# Autodesk Inventor assembly: Harbor Freight 10 in Wheel
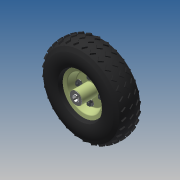
[picture p0: Inventor's stored thumbnail of the model, 180x180]
Saved by Autodesk Inventor 2018 (Build 220112000, 112)
## iProperties
Created: 2017-12-16
Part Number: Harbor Freight 10 in Wheel
Document SubType Name: Assembly
Designer: David
Author: David
## Documents named in this file (8)
- C:\Users\David\Documents\Inventor\Master\RC Car\Harbor Freight 10 in Wheel\Harbor Freight 10 in Wheel.iam
- C:\Users\David\Documents\Inventor\Master\RC Car\Harbor Freight 10 in Wheel\Hub Outer.ipt
- C:\Users\David\Documents\Inventor\Master\RC Car\Harbor Freight 10 in Wheel\Bolt M8x14mm.ipt
- C:\Users\David\Documents\Inventor\Master\RC Car\Harbor Freight 10 in Wheel\Nut M8.ipt
- C:\Users\David\Documents\Inventor\Master\RC Car\Harbor Freight 10 in Wheel\Washer Flat M8.ipt
- C:\Users\David\Documents\Inventor\Master\RC Car\Harbor Freight 10 in Wheel\Tire.ipt
- C:\Users\David\Documents\Inventor\Master\RC Car\Harbor Freight 10 in Wheel\Bearing.ipt
- C:\Users\David\Documents\Inventor\Master\RC Car\Harbor Freight 10 in Wheel\Hub Inner No Holes.ipt
## Components (21 placed, 7 different names)
1. Hub Inner No Holes:1 — Mate:1, Mate:2, Mate:3, Insert:13, Insert:14, Insert:15, Insert:16, Mate:6, Mate:7, Mate:8
2. Hub Outer:1 — Mate:1, Mate:2, Mate:3, Mate:4, Mate:9
3. Bolt M8x14mm:1 — Insert:1
4. Nut M8:1 — Insert:3
5. Washer Flat M8:1 — Insert:2, Insert:3, Insert:14
6. Washer Flat M8:2 — Insert:1, Insert:2
7. Bolt M8x14mm:2
8. Nut M8:2
9. Washer Flat M8:3 — Insert:13
10. Washer Flat M8:4
11. Bolt M8x14mm:3
12. Nut M8:3
13. Washer Flat M8:5 — Insert:15
14. Washer Flat M8:6
15. Bolt M8x14mm:4
16. Nut M8:4
17. Washer Flat M8:7 — Insert:16
18. Washer Flat M8:8
19. Tire:1 — Mate:4, Mate:5
20. Bearing:1 — Mate:6, Mate:8
21. Bearing:2 — Mate:7, Mate:9
## Relationships (25: Insert 16, Mate 9)
- Mate:1: Hub Inner No Holes:1 ↔ Hub Outer:1
- Mate:2: Hub Inner No Holes:1 ↔ Hub Outer:1
- Mate:3: Hub Inner No Holes:1 ↔ Hub Outer:1
- Insert:1: Bolt M8x14mm:1 ↔ Washer Flat M8:2
- Insert:2 (3.048 mm): Washer Flat M8:1 ↔ Washer Flat M8:2
- Insert:3: Nut M8:1 ↔ Washer Flat M8:1
- [Insert]: Bolt M8x14mm:2 ↔ Washer Flat M8:4
- [Insert] (3.048 mm): Washer Flat M8:3 ↔ Washer Flat M8:4
- [Insert]: Nut M8:2 ↔ Washer Flat M8:3
- [Insert]: Bolt M8x14mm:3 ↔ Washer Flat M8:6
- [Insert] (3.048 mm): Washer Flat M8:5 ↔ Washer Flat M8:6
- [Insert]: Nut M8:3 ↔ Washer Flat M8:5
- [Insert]: Bolt M8x14mm:4 ↔ Washer Flat M8:8
- [Insert] (3.048 mm): Washer Flat M8:7 ↔ Washer Flat M8:8
- [Insert]: Nut M8:4 ↔ Washer Flat M8:7
- Insert:13: Hub Inner No Holes:1 ↔ Washer Flat M8:3
- Insert:14: Hub Inner No Holes:1 ↔ Washer Flat M8:1
- Insert:15: Hub Inner No Holes:1 ↔ Washer Flat M8:5
- Insert:16: Hub Inner No Holes:1 ↔ Washer Flat M8:7
- Mate:4: Hub Outer:1 ↔ Tire:1
- Mate:5: Tire:1
- Mate:6: Hub Inner No Holes:1 ↔ Bearing:1
- Mate:7: Hub Inner No Holes:1 ↔ Bearing:2
- Mate:8: Hub Inner No Holes:1 ↔ Bearing:1
- Mate:9: Hub Outer:1 ↔ Bearing:2
## Named parameters: d6_d3 = 0 mm, d7_d4 = 3.048 mm, d8_d5 = 0 mm, d9_d3 = 0 mm, d10_d4 = 3.048 mm, d11_d5 = 0 mm, d12_d3 = 0 mm, d13_d4 = 3.048 mm, d14_d5 = 0 mm
